# Autodesk Inventor assembly: 72-7-3664_angle 65
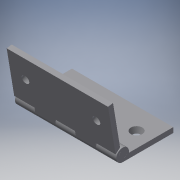
[picture p0: Inventor's stored thumbnail of the model, 180x180]
Saved by Autodesk Inventor 2016 (Build 200138000, 138)
## iProperties
Company: TraceParts S.A.
Created: 2018-11-02
Part Number: 72-7-3664_angle 65
Checked By: TraceParts S.A.
Catalog Web Link: www.traceparts.com
Document SubType Name: Assembly
Designer: TraceParts
material: brass
SUPPLIER: PINET
finish: raw
DESIGN: Brass hinges - 6 holes A
REFERENCE: 72-7-3664
TraceParts.PartVersion: 1.0.2
TraceParts.PartStatus: Published
TraceParts.PartNumber: 90-18062018-051905
TraceParts.PartLanguage: en
TraceParts.InstanceId: 90-18062018-051905E1KTYCC0X2J4WXGENV6BBILPD
TraceParts.PartTitle: Brass hinges - 6 holes A
TRACEPARTS: TRACEPARTS
TraceParts.ClassPath: PINET:/F_PINET/90-18062018-051905
Author: TraceParts
## Documents named in this file (3)
- C:\Users\hovm\Desktop\DaoCM's project\79748945-9-72-7-3664\72-7-3664_angle 65.iam
- C:\Users\hovm\Desktop\DaoCM's project\79748945-9-72-7-3664\72-7-3664_01.ipt
- C:\Users\hovm\Desktop\DaoCM's project\79748945-9-72-7-3664\72-7-3664_02.ipt
## Components (2 placed, 2 different names)
1. 72-7-3664_01:1 — Mate:1, Flush:1, Angle:1
2. 72-7-3664_02:1 — Mate:1, Flush:1, Angle:1
## Relationships (3: Mate 1, Flush 1, Angle 1)
- Mate:1: 72-7-3664_01:1 ↔ 72-7-3664_02:1
- Flush:1: 72-7-3664_01:1 ↔ 72-7-3664_02:1
- Angle:1 (80.5 deg): 72-7-3664_01:1 ↔ 72-7-3664_02:1
